# Autodesk Inventor assembly: shield_box
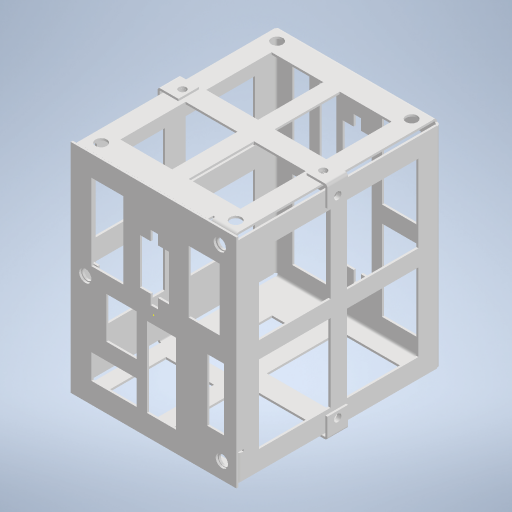
[picture p0: Inventor's stored thumbnail of the model, 512x512]
Saved by Autodesk Inventor 2023 (Build 270158000, 158)
## iProperties
Created: 2023-04-07
Part Number: shield_box
Document SubType Name: Assembly
Designer: 310611102
Author: 310611102
## Documents named in this file (4)
- C:\Users\310611102\Documents\Inventor\SSR\avionics_2023ver\electronics\shield box\shield_box.iam
- C:\Users\310611102\Documents\Inventor\SSR\avionics_2023ver\electronics\shield box\box.ipt
- C:\Users\310611102\Documents\Inventor\SSR\avionics_2023ver\electronics\shield box\cap.ipt
- C:\Users\310611102\Documents\Inventor\SSR\avionics_2023ver\electronics\shield box\joint.ipt
## Components (6 placed, 3 different names)
1. box:1 — Mate:1, Mate:2, Mate:3, Insert:1, Insert:2, Insert:3, Insert:4, Insert:6, Insert:7, Insert:8, Insert:9
2. cap:1 — Mate:1, Mate:2, Mate:3
3. joint:1 — Insert:1, Insert:2
4. joint:2 — Insert:3, Insert:4
5. joint:3 — Insert:6, Insert:7
6. joint:4 — Insert:8, Insert:9
## Relationships (11: Insert 8, Mate 3)
- Mate:1: box:1 ↔ cap:1
- Mate:2: box:1 ↔ cap:1
- Mate:3: box:1 ↔ cap:1
- Insert:1: box:1 ↔ joint:1
- Insert:2: box:1 ↔ joint:1
- Insert:3: box:1 ↔ joint:2
- Insert:4: box:1 ↔ joint:2
- Insert:6: box:1 ↔ joint:3
- Insert:7: box:1 ↔ joint:3
- Insert:8: box:1 ↔ joint:4
- Insert:9: box:1 ↔ joint:4
